# Autodesk Inventor assembly: shaft_with_components
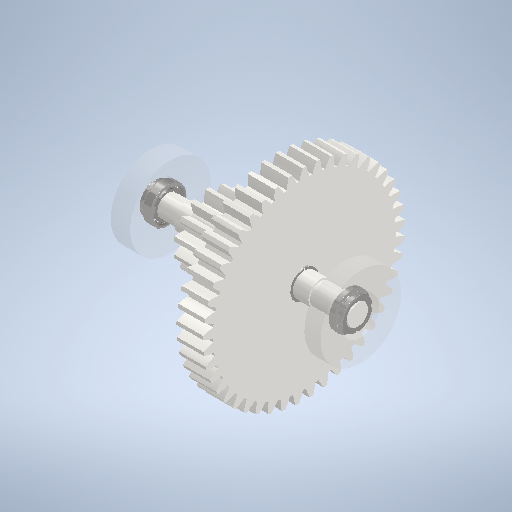
[picture p0: Inventor's stored thumbnail of the model, 512x512]
Saved by Autodesk Inventor 2025 (Build 290162010, 162A)
## iProperties
Created: 2024-06-04
Part Number: shaft_with_components
Document SubType Name: Assembly
Designer: Igor
Author: Igor
## Documents named in this file (12)
- C:\Users\Igor\Desktop\shaft_with_components.iam
- C:\Users\Igor\Documents\Inventor\wał.iam
- C:\Users\Igor\Documents\zebatka_duza.ipt
- C:\Users\Igor\Documents\zebatka_mala.ipt
- C:\Users\Igor\Documents\Złożenie\Design Accelerator\Łożysko1.iam
- C:\Users\Igor\Documents\Złożenie\Design Accelerator\Łożysko2.iam
- C:\Users\Igor\Documents\Inventor\Content Center Files\R2025\pl-PL\ISO 464\ISO 464 - 50.ipt
- C:\Users\Igor\Documents\Inventor\Content Center Files\R2025\pl-PL\ISO 464\ISO 464 - 47.ipt
- C:\Users\Igor\Documents\Inventor\Content Center Files\R2025\pl-PL\DIN 981\DIN 981 - KM 8.ipt
- C:\Users\Igor\Documents\Inventor\Content Center Files\R2025\pl-PL\DIN 5406 Type MB_MBL (- DIN 981)\DIN 5406 - MB8.ipt
- C:\Users\Igor\Documents\Część10.ipt
- C:\Users\Igor\Documents\Część11.ipt
## Components (14 placed, 10 different names)
1. wał:1 [sub-assembly] — Zestawiające:1, Zestawiające:2, Zestawiające:3, Zestawiające:4, Zestawiające:5, Zestawiające:6, Zestawiające:7, Zestawiające:8, Zestawiające:9, Zestawiające:10, Zestawiające:11, Zestawiające:12
2. Przekładnia walcowa1:1 — Zestawiające:3, Zestawiające:4, Wstawiające:1, Wstawiające:3
3. Przekładnia walcowa2:1 — Zestawiające:1, Zestawiające:2, Wstawiające:2
4. Łożysko:1 [sub-assembly] — Zestawiające:5
5. Łożysko:2 [sub-assembly] — Zestawiające:6
6. ISO 464 50:2 — Wstawiające:1
7. ISO 464 47:1 — Wstawiające:2
8. ISO 464 50:3 — Wstawiające:3
9. DIN 981 KM 8:1 — Zestawiające:8
10. DIN 981 KM 8:2 — Zestawiające:10
11. DIN 5406 Typ MB/MBL (->DIN 981) MB8:1 — Zestawiające:7
12. DIN 5406 Typ MB/MBL (->DIN 981) MB8:2 — Zestawiające:9
13. Korpus:1 — Zestawiające:11
14. Część11:1 — Zestawiające:12
## Relationships (15: Mate 12, Insert 3)
- Zestawiające:1 [Mate]: wał:1 ↔ Przekładnia walcowa2:1
- Zestawiające:2 [Mate]: wał:1 ↔ Przekładnia walcowa2:1
- Zestawiające:3 [Mate]: wał:1 ↔ Przekładnia walcowa1:1
- Zestawiające:4 [Mate] (30 mm): wał:1 ↔ Przekładnia walcowa1:1
- Zestawiające:5 [Mate]: wał:1 ↔ Łożysko:1
- Zestawiające:6 [Mate]: wał:1 ↔ Łożysko:2
- Wstawiające:1 [Insert]: Przekładnia walcowa1:1 ↔ ISO 464 50:2
- Wstawiające:2 [Insert]: Przekładnia walcowa2:1 ↔ ISO 464 47:1
- Wstawiające:3 [Insert]: Przekładnia walcowa1:1 ↔ ISO 464 50:3
- Zestawiające:7 [Mate]: wał:1 ↔ DIN 5406 Typ MB/MBL (->DIN 981) MB8:1
- Zestawiające:8 [Mate]: wał:1 ↔ DIN 981 KM 8:1
- Zestawiające:9 [Mate]: wał:1 ↔ DIN 5406 Typ MB/MBL (->DIN 981) MB8:2
- Zestawiające:10 [Mate]: wał:1 ↔ DIN 981 KM 8:2
- Zestawiające:11 [Mate]: wał:1 ↔ Korpus:1
- Zestawiające:12 [Mate]: wał:1 ↔ Część11:1
